# Autodesk Inventor assembly: Keilverbindung
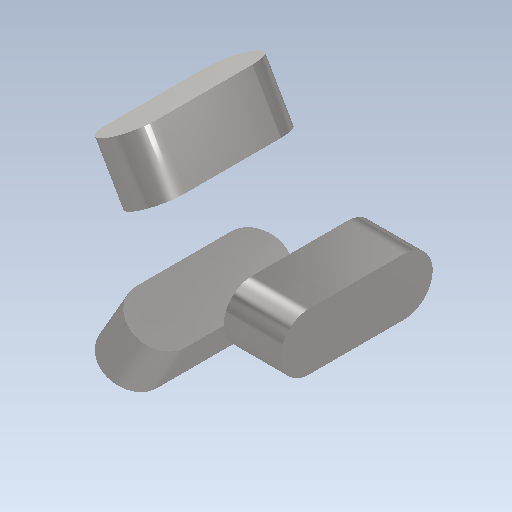
[picture p0: Inventor's stored thumbnail of the model, 512x512]
Saved by Autodesk Inventor 2021 (Build 250183000, 183)
## iProperties
ClientObjectVersion: 1
Created: 2021-01-25
Part Number: Keilverbindung
Document SubType Name: Assembly
Designer: Jaro Machnow
Author: Jaro Machnow
## Documents named in this file (2)
- C:\Users\Jaro Machnow\Documents\Vault\Gruppen\Gruppe 2\Entwurf\Amphibienfahrzeug\Wechsel zwischen Land und Wasser\Mechanik_zum_Wechseln\Wechselmechnanik\Konstruktions-Assistent\Keilverbindung2.iam
- C:\Users\Jaro Machnow\Documents\Inventor\Content Center Files\R2021\de-DE\DIN 6885-1 A\DIN 6885 - A 3 x 3 x 8.ipt
## Components (3 placed, 1 different names)
1. DIN 6885-1 A A 3 x 3 x 8:1
2. DIN 6885-1 A A 3 x 3 x 8:2
3. DIN 6885-1 A A 3 x 3 x 8:3
## Component patterns: (3 elements, first: DIN 6885-1 A A 3 x 3 x 8:1)
